# Autodesk Inventor assembly: 小装甲板装配
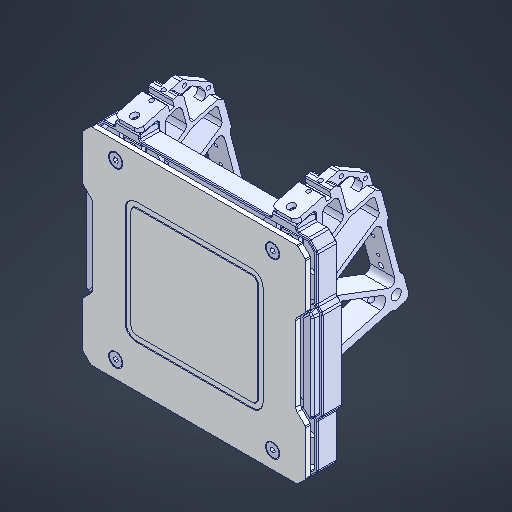
[picture p0: Inventor's stored thumbnail of the model, 512x512]
Saved by Autodesk Inventor 2025 (Build 290162000, 162)
## iProperties
Created: 2025-12-22
Part Number: 小装甲板装配
Document SubType Name: Assembly
Designer: XH
Author: XH
## Documents named in this file (3)
- C:\1A_Engineering_files\RCInventor\铝件版本\裁判系统\小装甲板装配.iam
- C:\1A_Engineering_files\RCInventor\铝件版本\RoboMaster 装甲模块 AM02 2019.ipt
- C:\1A_Engineering_files\RCInventor\铝件版本\RoboMaster 装甲支撑架A型 2019.ipt
## Components (3 placed, 2 different names)
1. RoboMaster 装甲模块 AM02 2019:1 — 配合:1, 配合:2, 配合:3, 配合:4
2. RoboMaster 装甲支撑架A型 2019:1 — 配合:1, 配合:2
3. RoboMaster 装甲支撑架A型 2019:2 — 配合:3, 配合:4
## Relationships (4: Mate 4)
- 配合:1 [Mate]: RoboMaster 装甲模块 AM02 2019:1 ↔ RoboMaster 装甲支撑架A型 2019:1
- 配合:2 [Mate]: RoboMaster 装甲模块 AM02 2019:1 ↔ RoboMaster 装甲支撑架A型 2019:1
- 配合:3 [Mate]: RoboMaster 装甲模块 AM02 2019:1 ↔ RoboMaster 装甲支撑架A型 2019:2
- 配合:4 [Mate]: RoboMaster 装甲模块 AM02 2019:1 ↔ RoboMaster 装甲支撑架A型 2019:2
